# Autodesk Inventor assembly: FE-00014-02
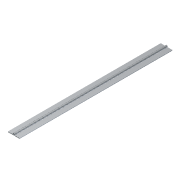
[picture p0: Inventor's stored thumbnail of the model, 180x180]
Saved by Autodesk Inventor 2012 (Build 160160000, 160)
## iProperties
Company: FIRST
Created: 2008-05-25
Part Number: FE-00014-02
Document SubType Name: Assembly
Designer: dfoster
Description: Hinge
Title: Hinge
Author: dfoster
## Documents named in this file (2)
- C:\Data Folder\FRC 2012 Field\Components\FE-00014-02.iam
- C:\Data Folder\FRC 2012 Field\Components\FE-00014-02.ipt
## Components (2 placed, 1 different names)
1. FE-00014-02:1 — Mate:1, Mate:2, Angle:1
2. FE-00014-02:2 — Mate:1, Mate:2, Angle:1
## Relationships (3: Mate 2, Angle 1)
- Mate:1: FE-00014-02:1 ↔ FE-00014-02:2
- Mate:2: FE-00014-02:1 ↔ FE-00014-02:2
- Angle:1 (0 deg): FE-00014-02:1 ↔ FE-00014-02:2
